# Autodesk Inventor assembly: HeatSink-sheet-assembly-H14mm
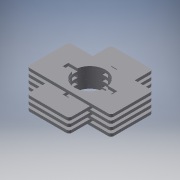
[picture p0: Inventor's stored thumbnail of the model, 180x180]
Saved by Autodesk Inventor 2017 (Build 210142000, 142)
## iProperties
Created: 2022-06-02
Part Number: HeatSink-sheet-assembly-H14mm
Document SubType Name: Assembly
Designer: Nikita
Author: Nikita
## Documents named in this file (2)
- C:\Users\Nikita\Documents\GitHub\mesoSPIM-bt-hardware\Benchtop\custom-parts\galvo-assembly\15mm-galvo(Thorlabs-QS15)-mount\HeatSink-sheet-assembly-H14mm.iam
- C:\Users\Nikita\Documents\GitHub\mesoSPIM-bt-hardware\Benchtop\custom-parts\galvo-assembly\15mm-galvo(Thorlabs-QS15)-mount\HeatSink-sheet-H2mm.ipt
## Components (7 placed, 1 different names)
1. HeatSink-sheet-H2mm:1 — Insert:1
2. HeatSink-sheet-H2mm:2 — Insert:1, Insert:2
3. HeatSink-sheet-H2mm:3 — Insert:2, Insert:3
4. HeatSink-sheet-H2mm:4 — Insert:3, Insert:4
5. HeatSink-sheet-H2mm:5 — Insert:4, Insert:5
6. HeatSink-sheet-H2mm:6 — Insert:5, Insert:6
7. HeatSink-sheet-H2mm:7 — Insert:6
## Relationships (6: Insert 6)
- Insert:1: HeatSink-sheet-H2mm:1 ↔ HeatSink-sheet-H2mm:2
- Insert:2: HeatSink-sheet-H2mm:2 ↔ HeatSink-sheet-H2mm:3
- Insert:3: HeatSink-sheet-H2mm:3 ↔ HeatSink-sheet-H2mm:4
- Insert:4: HeatSink-sheet-H2mm:4 ↔ HeatSink-sheet-H2mm:5
- Insert:5: HeatSink-sheet-H2mm:5 ↔ HeatSink-sheet-H2mm:6
- Insert:6: HeatSink-sheet-H2mm:6 ↔ HeatSink-sheet-H2mm:7
